# Autodesk Inventor assembly: detectionAxis
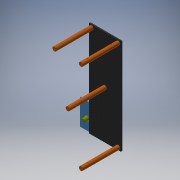
[picture p0: Inventor's stored thumbnail of the model, 180x180]
Saved by Autodesk Inventor 2016 (Build 200138000, 138)
## iProperties
Created: 2016-03-13
Part Number: detectionAxis
Document SubType Name: Assembly
Designer: sims01
Author: sims01
## Documents named in this file (6)
- H:\Documents\LSFM_3\setup\mechanical\design\lsfm3_mechDesign\detectionAxis.iam
- H:\Documents\LSFM_3\setup\mechanical\design\lsfm3_mechDesign\300x900mmBreadboard.ipt
- H:\Documents\LSFM_3\setup\mechanical\design\lsfm3_mechDesign\detectionObjAssembly.iam
- H:\Documents\LSFM_3\setup\mechanical\design\lsfm3_mechDesign\sCMOSassembly.iam
- H:\Documents\LSFM_3\setup\mechanical\design\lsfm3_mechDesign\50.8mmCageRod.ipt
- H:\Documents\LSFM_3\setup\mechanical\design\lsfm3_mechDesign\360mmPost.iam
## Components (11 placed, 5 different names)
1. 300x900mmBreadboard:1 — Rigid:7, Rigid:8, Rigid:9, Rigid:10, Rigid:11
2. sCMOSassembly:1 [sub-assembly]
3. 50.8mmCageRod:1
4. 50.8mmCageRod:2
5. 50.8mmCageRod:3
6. 50.8mmCageRod:4
7. 360mmPost:1 [sub-assembly] — Rigid:9
8. 360mmPost:2 [sub-assembly] — Rigid:10
9. 360mmPost:3 [sub-assembly] — Rigid:8
10. 360mmPost:4 [sub-assembly] — Rigid:7
11. detectionObjAssembly:1 [sub-assembly] — Rigid:11
## Relationships (5: WeldJoint 5)
- Rigid:7 [WeldJoint]: 300x900mmBreadboard:1 ↔ 360mmPost:4
- Rigid:8 [WeldJoint]: 300x900mmBreadboard:1 ↔ 360mmPost:3
- Rigid:9 [WeldJoint]: 300x900mmBreadboard:1 ↔ 360mmPost:1
- Rigid:10 [WeldJoint]: 300x900mmBreadboard:1 ↔ 360mmPost:2
- Rigid:11 [WeldJoint]: 300x900mmBreadboard:1 ↔ detectionObjAssembly:1
